# Autodesk Inventor assembly: pvcRails
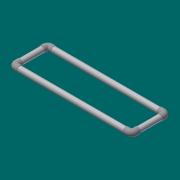
[picture p0: Inventor's stored thumbnail of the model, 180x180]
Saved by Autodesk Inventor 2016 (Build 200138000, 138)
## iProperties
Created: 2016-02-10
Part Number: pvcRails
Document SubType Name: Assembly
Designer: Sawaiz
Author: Sawaiz
## Documents named in this file (4)
- C:\Users\Sawaiz\OneDrive\projects\modularRICH\rails\pvcRails.iam
- C:\Users\Sawaiz\OneDrive\projects\modularRICH\rails\longRail.ipt
- C:\Users\Sawaiz\OneDrive\projects\modularRICH\rails\2inPvcElbow.ipt
- C:\Users\Sawaiz\OneDrive\projects\modularRICH\rails\railSeperator.ipt
## Components (8 placed, 3 different names)
1. longRail:1 — Mate:5, Mate:6, Mate:13
2. longRail:2 — Mate:1, Mate:2, Mate:9, Mate:12
3. 2inPvcElbow:1 — Mate:1, Mate:8, Mate:9
4. 2inPvcElbow:2 — Mate:2, Mate:3, Mate:11, Mate:12
5. 2inPvcElbow:3 — Mate:4, Mate:5, Mate:10, Mate:13
6. 2inPvcElbow:4 — Mate:6, Mate:7, Mate:14
7. railSeperator:1 — Mate:7, Mate:8, Mate:14
8. railSeperator:2 — Mate:3, Mate:4, Mate:10, Mate:11
## Relationships (14: Mate 14)
- Mate:1: longRail:2 ↔ 2inPvcElbow:1
- Mate:2: longRail:2 ↔ 2inPvcElbow:2
- Mate:3: 2inPvcElbow:2 ↔ railSeperator:2
- Mate:4: 2inPvcElbow:3 ↔ railSeperator:2
- Mate:5: longRail:1 ↔ 2inPvcElbow:3
- Mate:6: longRail:1 ↔ 2inPvcElbow:4
- Mate:7: 2inPvcElbow:4 ↔ railSeperator:1
- Mate:8: 2inPvcElbow:1 ↔ railSeperator:1
- Mate:9: longRail:2 ↔ 2inPvcElbow:1
- Mate:10: 2inPvcElbow:3 ↔ railSeperator:2
- Mate:11: 2inPvcElbow:2 ↔ railSeperator:2
- Mate:12: longRail:2 ↔ 2inPvcElbow:2
- Mate:13: longRail:1 ↔ 2inPvcElbow:3
- Mate:14: 2inPvcElbow:4 ↔ railSeperator:1
